# Autodesk Inventor assembly: Leg_left
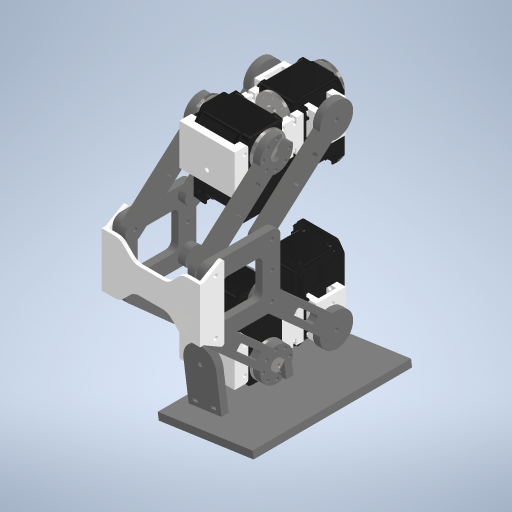
[picture p0: Inventor's stored thumbnail of the model, 512x512]
Saved by Autodesk Inventor 2024.3 (Build 283343000, 343)
## iProperties
Created: 2024-09-18
Part Number: Leg_left
Document SubType Name: Assembly
Designer: 구지현
Author: 구지현
## Documents named in this file (20)
- C:\Users\구지현\Desktop\19th_intern_kdy_fight_robot\부품\Lower_Body\Leg\Leg_left.iam
- C:\Users\구지현\Desktop\19th_intern_kdy_fight_robot\부품\Lower_Body\Leg\Back_Ankle.ipt
- C:\Users\구지현\Desktop\19th_intern_kdy_fight_robot\부품\Lower_Body\Leg\Front_Ankle.ipt
- C:\Users\구지현\Desktop\19th_intern_kdy_fight_robot\부품\Lower_Body\Leg\Knee.ipt
- C:\Users\구지현\Desktop\19th_intern_kdy_fight_robot\부품\Lower_Body\Leg\Knee_Covers.ipt
- C:\Users\구지현\Desktop\19th_intern_kdy_fight_robot\부품\Lower_Body\Leg\Leg_Connection_Parts_Back.ipt
- C:\Users\구지현\Desktop\19th_intern_kdy_fight_robot\부품\Lower_Body\Leg\Leg_Connection_Parts_Front.ipt
- C:\Users\구지현\Desktop\19th_intern_kdy_fight_robot\부품\Lower_Body\Leg\Leg_Foot_Connection_Parts.ipt
- C:\Users\구지현\Desktop\19th_intern_kdy_fight_robot\부품\Lower_Body\Leg\Link_Fixation_Connector.ipt
- C:\Users\구지현\Desktop\19th_intern_kdy_fight_robot\부품\Lower_Body\Leg\Vertical_Fixation_Set.iam
- C:\Users\구지현\Desktop\19th_intern_kdy_fight_robot\부품\Lower_Body\Leg\Link_Fixation_Connector_MIR.ipt
- Link_Fixation_Connector_left_left.ipt
- C:\Users\구지현\Desktop\19th_intern_kdy_fight_robot\부품\Lower_Body\Leg\Foot_MIR.ipt
- C:\Users\구지현\Desktop\19th_intern_kdy_fight_robot\부품\Lower_Body\Leg\Link_Fixation_Connector_MIR1.ipt
- C:\Users\구지현\Desktop\19th_intern_kdy_fight_robot\부품\Lower_Body\Leg\Link_Fixation_Connector_MIR_MIR.ipt
- C:\Users\구지현\Desktop\19th_intern_kdy_fight_robot\부품\ROBOTIS(Inventor 2024 ver.)\혼\64-106Horn.ipt
- C:\Users\구지현\Desktop\19th_intern_kdy_fight_robot\부품\ROBOTIS(Inventor 2024 ver.)\다이나믹셀\MX-106T+idle.ipt.iam
- C:\Users\구지현\Desktop\19th_intern_kdy_fight_robot\부품\ROBOTIS(Inventor 2024 ver.)\다이나믹셀\MX-64T+idle.ipt.iam
- MX-106T+idle.ipt
- MX-64T+idle.ipt
## Components (30 placed, 16 different names)
1. Back_Ankle:1 — 플러쉬:14, 각도:9, 삽입:37, 삽입:40
2. Knee:1 — 삽입:18, 삽입:19, 플러쉬:4, 플러쉬:5, 삽입:23, 삽입:28, 삽입:29, 삽입:33
3. Knee_Covers:1 — 삽입:28, 삽입:29, 삽입:30, 삽입:31
4. Leg_Connection_Parts_Back:1 — 각도:5, 플러쉬:1, 각도:6, 메이트:18, 플러쉬:3, 삽입:18
5. Leg_Connection_Parts_Front:1 — 각도:3, 각도:4, 각도:7, 플러쉬:2, 삽입:21, 메이트:46, 메이트:47
6. Leg_Foot_Connection_Parts:1 — 삽입:35, 메이트:50, 메이트:51
7. Link_Fixation_Connector:1 — 메이트:18
8. Vertical_Fixation_Set:1 [sub-assembly] — 플러쉬:17, 메이트:52, 메이트:53, 메이트:54, 메이트:55
9. Leg_Connection_Parts_Front:2 — 각도:3, 각도:4, 각도:6, 플러쉬:3, 삽입:19
10. Link_Fixation_Connector_left_left:1 — 메이트:19, 메이트:56, 메이트:57
11. Leg_Connection_Parts_Back:2 — 각도:5, 플러쉬:1, 각도:7, 메이트:19, 플러쉬:2, 삽입:20
12. Knee:2 — 삽입:20, 삽입:21, 플러쉬:4, 플러쉬:5, 삽입:22, 삽입:30, 삽입:31, 삽입:32
13. Leg_Connection_Parts_Front:3 — 삽입:22, 플러쉬:6, 플러쉬:11, 각도:8, 메이트:48, 메이트:49
14. Leg_Connection_Parts_Front:4 — 삽입:23, 플러쉬:6, 플러쉬:13
15. Leg_Connection_Parts_Back:3 — 플러쉬:11, 각도:8, 삽입:32, 플러쉬:12, 메이트:45
16. Leg_Connection_Parts_Back:4 — 삽입:33, 플러쉬:12, 플러쉬:13, 메이트:41
17. Front_Ankle:2 — 삽입:35, 플러쉬:14, 각도:9, 삽입:36
18. Foot_left:1 — 삽입:36, 삽입:37
19. Leg_Foot_Connection_Parts:3
20. Vertical_Fixation_Set:3 [sub-assembly] — 플러쉬:17, 삽입:43, 삽입:44
21. Link_Fixation_Connector_left_right_top:1 — 메이트:41
22. Link_Fixation_Connector_left_left_top:1 — 메이트:45
23. 64-106Horn:1 — 메이트:48, 메이트:49, 삽입:41
24. 64-106Horn:2 — 메이트:46, 메이트:47, 삽입:38
25. MX-106T+idle.ipt:1 [sub-assembly] — 삽입:38, 메이트:50, 메이트:51, 메이트:52, 메이트:53, 플러쉬:18, 각도:10
26. MX-106T+idle.ipt:2 [sub-assembly] — 삽입:41, 플러쉬:18, 각도:10
27. 64-106Horn:3 — 삽입:42
28. 64-106Horn:4 — 삽입:39, 삽입:40
29. MX-64T+idle.ipt:1 [sub-assembly] — 삽입:42, 삽입:43, 삽입:44
30. MX-64T+idle.ipt:2 [sub-assembly] — 삽입:39, 메이트:54, 메이트:55, 메이트:56, 메이트:57
## Relationships (58: Insert 22, Mate 16, Flush 12, Angle 8)
- 각도:3 [Angle] (0 deg): Leg_Connection_Parts_Front:1 ↔ Leg_Connection_Parts_Front:2
- 각도:4 [Angle] (0 deg): Leg_Connection_Parts_Front:1 ↔ Leg_Connection_Parts_Front:2
- 각도:5 [Angle] (0 deg): Leg_Connection_Parts_Back:1 ↔ Leg_Connection_Parts_Back:2
- 플러쉬:1 [Flush]: Leg_Connection_Parts_Back:1 ↔ Leg_Connection_Parts_Back:2
- 각도:6 [Angle] (0 deg): Leg_Connection_Parts_Back:1 ↔ Leg_Connection_Parts_Front:2
- 각도:7 [Angle] (0 deg): Leg_Connection_Parts_Front:1 ↔ Leg_Connection_Parts_Back:2
- 메이트:18 [Mate]: Leg_Connection_Parts_Back:1 ↔ Link_Fixation_Connector:1
- 메이트:19 [Mate]: Link_Fixation_Connector_left_left:1 ↔ Leg_Connection_Parts_Back:2
- 플러쉬:2 [Flush]: Leg_Connection_Parts_Front:1 ↔ Leg_Connection_Parts_Back:2
- 플러쉬:3 [Flush]: Leg_Connection_Parts_Back:1 ↔ Leg_Connection_Parts_Front:2
- 삽입:18 [Insert]: Knee:1 ↔ Leg_Connection_Parts_Back:1
- 삽입:19 [Insert]: Knee:1 ↔ Leg_Connection_Parts_Front:2
- 삽입:20 [Insert]: Leg_Connection_Parts_Back:2 ↔ Knee:2
- 삽입:21 [Insert]: Leg_Connection_Parts_Front:1 ↔ Knee:2
- 플러쉬:4 [Flush]: Knee:1 ↔ Knee:2
- 플러쉬:5 [Flush]: Knee:1 ↔ Knee:2
- 삽입:22 [Insert]: Knee:2 ↔ Leg_Connection_Parts_Front:3
- 삽입:23 [Insert]: Knee:1 ↔ Leg_Connection_Parts_Front:4
- 플러쉬:6 [Flush]: Leg_Connection_Parts_Front:3 ↔ Leg_Connection_Parts_Front:4
- 삽입:28 [Insert]: Knee:1 ↔ Knee_Covers:1
- 삽입:29 [Insert]: Knee:1 ↔ Knee_Covers:1
- 삽입:30 [Insert]: Knee_Covers:1 ↔ Knee:2
- 삽입:31 [Insert]: Knee_Covers:1 ↔ Knee:2
- 플러쉬:11 [Flush]: Leg_Connection_Parts_Front:3 ↔ Leg_Connection_Parts_Back:3
- 각도:8 [Angle] (0 deg): Leg_Connection_Parts_Front:3 ↔ Leg_Connection_Parts_Back:3
- 삽입:32 [Insert]: Knee:2 ↔ Leg_Connection_Parts_Back:3
- 삽입:33 [Insert]: Knee:1 ↔ Leg_Connection_Parts_Back:4
- 플러쉬:12 [Flush]: Leg_Connection_Parts_Back:3 ↔ Leg_Connection_Parts_Back:4
- 플러쉬:13 [Flush]: Leg_Connection_Parts_Front:4 ↔ Leg_Connection_Parts_Back:4
- 삽입:35 [Insert]: Leg_Foot_Connection_Parts:1 ↔ Front_Ankle:2
- 플러쉬:14 [Flush]: Back_Ankle:1 ↔ Front_Ankle:2
- 각도:9 [Angle] (0 deg): Back_Ankle:1 ↔ Front_Ankle:2
- 삽입:36 [Insert]: Front_Ankle:2 ↔ Foot_left:1
- 삽입:37 [Insert]: Back_Ankle:1 ↔ Foot_left:1
- 플러쉬:17 [Flush]: Vertical_Fixation_Set:1 ↔ Vertical_Fixation_Set:3
- 메이트:41 [Mate]: Leg_Connection_Parts_Back:4 ↔ Link_Fixation_Connector_left_right_top:1
- 메이트:45 [Mate]: Leg_Connection_Parts_Back:3 ↔ Link_Fixation_Connector_left_left_top:1
- 메이트:46 [Mate]: Leg_Connection_Parts_Front:1 ↔ 64-106Horn:2
- 메이트:47 [Mate]: Leg_Connection_Parts_Front:1 ↔ 64-106Horn:2
- 메이트:48 [Mate]: Leg_Connection_Parts_Front:3 ↔ 64-106Horn:1
- 메이트:49 [Mate]: Leg_Connection_Parts_Front:3 ↔ 64-106Horn:1
- 삽입:38 [Insert]: 64-106Horn:2 ↔ MX-106T+idle.ipt:1
- 메이트:50 [Mate]: Leg_Foot_Connection_Parts:1 ↔ MX-106T+idle.ipt:1
- 메이트:51 [Mate]: Leg_Foot_Connection_Parts:1 ↔ MX-106T+idle.ipt:1
- 메이트:52 [Mate]: Vertical_Fixation_Set:1 ↔ MX-106T+idle.ipt:1
- 메이트:53 [Mate]: Vertical_Fixation_Set:1 ↔ MX-106T+idle.ipt:1
- 삽입:39 [Insert]: 64-106Horn:4 ↔ MX-64T+idle.ipt:2
- 삽입:40 [Insert]: Back_Ankle:1 ↔ 64-106Horn:4
- 메이트:54 [Mate]: Vertical_Fixation_Set:1 ↔ MX-64T+idle.ipt:2
- 메이트:55 [Mate]: Vertical_Fixation_Set:1 ↔ MX-64T+idle.ipt:2
- 메이트:56 [Mate]: Link_Fixation_Connector_left_left:1 ↔ MX-64T+idle.ipt:2
- 메이트:57 [Mate]: Link_Fixation_Connector_left_left:1 ↔ MX-64T+idle.ipt:2
- 삽입:41 [Insert]: 64-106Horn:1 ↔ MX-106T+idle.ipt:2
- 플러쉬:18 [Flush]: MX-106T+idle.ipt:1 ↔ MX-106T+idle.ipt:2
- 각도:10 [Angle] (0 deg): MX-106T+idle.ipt:1 ↔ MX-106T+idle.ipt:2
- 삽입:42 [Insert]: 64-106Horn:3 ↔ MX-64T+idle.ipt:1
- 삽입:43 [Insert]: Vertical_Fixation_Set:3 ↔ MX-64T+idle.ipt:1
- 삽입:44 [Insert]: Vertical_Fixation_Set:3 ↔ MX-64T+idle.ipt:1
